# Autodesk Inventor assembly: Joystick_Box
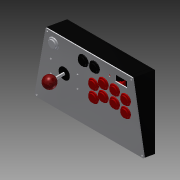
[picture p0: Inventor's stored thumbnail of the model, 180x180]
Saved by Autodesk Inventor 2013 (Build 170138000, 138)
## iProperties
Created: 2012-08-20
Part Number: Joystick_Box
Document SubType Name: Assembly
Designer: Brandon
Author: Brandon
## Documents named in this file (9)
- C:\Users\bbooth\Documents\GitHub\Pew-Pew-Stick\assemblies\Joystick_Box.iam
- C:\Users\bbooth\Documents\GitHub\Pew-Pew-Stick\parts\Panel_top.ipt
- C:\Users\bbooth\Documents\GitHub\Pew-Pew-Stick\parts\Panel_side.ipt
- C:\Users\bbooth\Documents\GitHub\Pew-Pew-Stick\parts\Panel_bottom.ipt
- C:\Users\bbooth\Documents\GitHub\Pew-Pew-Stick\parts\Panel_side_MIR.ipt
- C:\Users\bbooth\Documents\GitHub\Pew-Pew-Stick\parts\Panel_front.ipt
- C:\Users\bbooth\Documents\GitHub\Pew-Pew-Stick\parts\Panel_back.ipt
- C:\Users\bbooth\Documents\GitHub\Pew-Pew-Stick\parts\Sanwa_Joystick_JLF-TP-8YT.ipt
- C:\Users\bbooth\Documents\GitHub\Pew-Pew-Stick\parts\OBSF-30-B_button.ipt
## Components (18 placed, 8 different names)
1. Panel_top:1 — Flush:7, Insert:1, Insert:2, Insert:3, Insert:4, Insert:5, Insert:6, Insert:7, Insert:8, Insert:9, Insert:10, Insert:11, Insert:12, Mate:5, Mate:7
2. Panel_bottom:1 — Mate:1, Flush:1, Flush:2, Flush:3, Mate:2, Flush:4, Flush:5, Mate:4
3. Panel_side:2 — Mate:1, Flush:1, Flush:2, Flush:3
4. Panel_side_MIR:1 — Mate:2, Flush:4, Flush:5, Mate:3, Flush:6, Mate:6, Flush:8
5. Panel_front:1 — Mate:3, Mate:4, Flush:6, Flush:7
6. Panel_back:1 — Mate:5, Mate:6, Flush:8, Mate:7
7. Sanwa_Joystick_JLF-TP-8YT:1 — Insert:12
8. OBSF-30-B_button:1 — Insert:7
9. OBSF-30-B_button:2 — Insert:1
10. OBSF-30-B_button:3 — Insert:2
11. OBSF-30-B_button:4 — Insert:3
12. OBSF-30-B_button:5 — Insert:5
13. OBSF-30-B_button:6 — Insert:6
14. OBSF-30-B_button:7 — Insert:8
15. OBSF-30-B_button:8 — Insert:10
16. OBSF-30-B_button:9 — Insert:4
17. OBSF-30-B_button:10 — Insert:9
18. OBSF-30-B_button:11 — Insert:11
## Relationships (27: Insert 12, Flush 8, Mate 7)
- Mate:1: Panel_bottom:1 ↔ Panel_side:2
- Flush:1: Panel_bottom:1 ↔ Panel_side:2
- Flush:2: Panel_bottom:1 ↔ Panel_side:2
- Flush:3: Panel_bottom:1 ↔ Panel_side:2
- Mate:2: Panel_bottom:1 ↔ Panel_side_MIR:1
- Flush:4: Panel_bottom:1 ↔ Panel_side_MIR:1
- Flush:5: Panel_bottom:1 ↔ Panel_side_MIR:1
- Mate:3: Panel_side_MIR:1 ↔ Panel_front:1
- Mate:4: Panel_bottom:1 ↔ Panel_front:1
- Flush:6: Panel_side_MIR:1 ↔ Panel_front:1
- Flush:7: Panel_top:1 ↔ Panel_front:1
- Insert:1: Panel_top:1 ↔ OBSF-30-B_button:2
- Insert:2: Panel_top:1 ↔ OBSF-30-B_button:3
- Insert:3: Panel_top:1 ↔ OBSF-30-B_button:4
- Insert:4: Panel_top:1 ↔ OBSF-30-B_button:9
- Insert:5: Panel_top:1 ↔ OBSF-30-B_button:5
- Insert:6: Panel_top:1 ↔ OBSF-30-B_button:6
- Insert:7: Panel_top:1 ↔ OBSF-30-B_button:1
- Insert:8: Panel_top:1 ↔ OBSF-30-B_button:7
- Insert:9: Panel_top:1 ↔ OBSF-30-B_button:10
- Insert:10: Panel_top:1 ↔ OBSF-30-B_button:8
- Insert:11: Panel_top:1 ↔ OBSF-30-B_button:11
- Insert:12 (-0.2 mm): Panel_top:1 ↔ Sanwa_Joystick_JLF-TP-8YT:1
- Mate:5: Panel_top:1 ↔ Panel_back:1
- Mate:6: Panel_side_MIR:1 ↔ Panel_back:1
- Flush:8: Panel_side_MIR:1 ↔ Panel_back:1
- Mate:7: Panel_top:1 ↔ Panel_back:1
